# Autodesk Inventor assembly: WheelSuspension
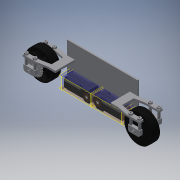
[picture p0: Inventor's stored thumbnail of the model, 180x180]
Saved by Autodesk Inventor 2017 (Build 210142000, 142)
## iProperties
Created: 2018-05-04
Part Number: WheelSuspension
Document SubType Name: Assembly
Designer: User
Author: User
## Documents named in this file (11)
- C:\Robotics\CAD\2018-19_CAD\Offseason\WheelSuspension.iam
- C:\Robotics\CAD\COTSParts\Fasteners\97345A207_316 STAINLESS STEEL SHOULDER SCREW.ipt
- C:\Robotics\CAD\COTSParts\Wheels\4in Wheel Intergreated Hub 8mm Rev2.ipt
- C:\Robotics\CAD\2016-17_CAD\Custom COTS\4inax.ipt
- C:\Robotics\CAD\2018-19_CAD\Offseason\WheelSuspensionHub.ipt
- C:\Robotics\CAD\COTSParts\Actobotics\535 parts\535198Bearing.25ID.5OD.ipt
- C:\Robotics\CAD\2018-19_CAD\Offseason\WheelandSprocketComboHub2.ipt
- C:\Robotics\CAD\COTSParts\Actobotics\615 parts\615106Sprocket.5inBore.25inPitch24Teeth.ipt
- C:\Robotics\CAD\2018-19_CAD\Offseason\WheelSuspensionFork.ipt
- C:\Robotics\CAD\2018-19_CAD\Offseason\SuspensionDrivePlate.ipt
- C:\Robotics\CAD\COTSParts\Rev\REV-41-1300HexMotor.ipt
## Components (30 placed, 10 different names)
1. 97345A207_316 STAINLESS STEEL SHOULDER SCREW:1 — Insert:3, Mate:3, Insert:11
2. 4in Wheel Intergreated Hub 8mm Rev2:1 — Insert:6
3. 4inax:1 — Insert:2
4. WheelSuspensionHub:1 — Insert:1, Insert:3, Mate:2, Insert:10
5. 535198Bearing.25ID.5OD:1 — Insert:1, Insert:2
6. WheelandSprocketComboHub2:1 — Insert:5, Insert:6, Insert:10
7. 615106Sprocket.5inBore.25inPitch24Teeth:1 — Insert:5
8. WheelSuspensionHub:2 — Insert:7, Insert:9
9. 97345A207_316 STAINLESS STEEL SHOULDER SCREW:2 — Insert:9, Mate:3, Insert:12
10. 535198Bearing.25ID.5OD:2 — Insert:7, Mate:2
11. WheelSuspensionFork:1 — Angle:1, Insert:11, Insert:12, Insert:13, Insert:14, Insert:27, Insert:28, Insert:31, Insert:34
12. 97345A207_316 STAINLESS STEEL SHOULDER SCREW:3 — Insert:13
13. 97345A207_316 STAINLESS STEEL SHOULDER SCREW:4 — Insert:14
14. 97345A207_316 STAINLESS STEEL SHOULDER SCREW:5
15. 4in Wheel Intergreated Hub 8mm Rev2:2
16. 4inax:2
17. WheelSuspensionHub:3
18. 535198Bearing.25ID.5OD:3
19. WheelandSprocketComboHub2:2
20. 615106Sprocket.5inBore.25inPitch24Teeth:2
21. WheelSuspensionHub:4
22. 97345A207_316 STAINLESS STEEL SHOULDER SCREW:6
23. 535198Bearing.25ID.5OD:4
24. WheelSuspensionFork:2 — Insert:29, Insert:30, Insert:32, Insert:33
25. 97345A207_316 STAINLESS STEEL SHOULDER SCREW:7
26. 97345A207_316 STAINLESS STEEL SHOULDER SCREW:8
27. SuspensionDrivePlate:1 — Insert:27, Insert:28, Insert:29, Insert:30
28. SuspensionDrivePlate:2 — Insert:31, Insert:32, Insert:33, Insert:34, Mate:6, Flush:1, Flush:2, Mate:7, Mate:8, Flush:3, Mate:10
29. REV-41-1300HexMotor:1 — Mate:8, Mate:9, Flush:3, Flush:4, Mate:10
30. REV-41-1300HexMotor:2 — Mate:7, Mate:9, Flush:4
## Relationships (46: Insert 32, Mate 9, Flush 4, Angle 1)
- Insert:1: WheelSuspensionHub:1 ↔ 535198Bearing.25ID.5OD:1
- Insert:2 (3.175 mm): 4inax:1 ↔ 535198Bearing.25ID.5OD:1
- Insert:3: 97345A207_316 STAINLESS STEEL SHOULDER SCREW:1 ↔ WheelSuspensionHub:1
- Insert:5: WheelandSprocketComboHub2:1 ↔ 615106Sprocket.5inBore.25inPitch24Teeth:1
- Insert:6: 4in Wheel Intergreated Hub 8mm Rev2:1 ↔ WheelandSprocketComboHub2:1
- Insert:7: WheelSuspensionHub:2 ↔ 535198Bearing.25ID.5OD:2
- Insert:9: WheelSuspensionHub:2 ↔ 97345A207_316 STAINLESS STEEL SHOULDER SCREW:2
- Mate:2: WheelSuspensionHub:1 ↔ 535198Bearing.25ID.5OD:2
- Mate:3 (63.5 mm): 97345A207_316 STAINLESS STEEL SHOULDER SCREW:1 ↔ 97345A207_316 STAINLESS STEEL SHOULDER SCREW:2
- Angle:1 (0 deg): WheelSuspensionFork:1
- Insert:10 (1.27 mm): WheelSuspensionHub:1 ↔ WheelandSprocketComboHub2:1
- Insert:11: 97345A207_316 STAINLESS STEEL SHOULDER SCREW:1 ↔ WheelSuspensionFork:1
- Insert:12: 97345A207_316 STAINLESS STEEL SHOULDER SCREW:2 ↔ WheelSuspensionFork:1
- Insert:13: WheelSuspensionFork:1 ↔ 97345A207_316 STAINLESS STEEL SHOULDER SCREW:3
- Insert:14: WheelSuspensionFork:1 ↔ 97345A207_316 STAINLESS STEEL SHOULDER SCREW:4
- [Insert]: WheelSuspensionHub:3 ↔ 535198Bearing.25ID.5OD:3
- [Insert] (3.175 mm): 4inax:2 ↔ 535198Bearing.25ID.5OD:3
- [Insert]: 97345A207_316 STAINLESS STEEL SHOULDER SCREW:5 ↔ WheelSuspensionHub:3
- [Insert]: WheelandSprocketComboHub2:2 ↔ 615106Sprocket.5inBore.25inPitch24Teeth:2
- [Insert]: 4in Wheel Intergreated Hub 8mm Rev2:2 ↔ WheelandSprocketComboHub2:2
- [Insert]: WheelSuspensionHub:4 ↔ 535198Bearing.25ID.5OD:4
- [Insert]: WheelSuspensionHub:4 ↔ 97345A207_316 STAINLESS STEEL SHOULDER SCREW:6
- [Mate]: WheelSuspensionHub:3 ↔ 535198Bearing.25ID.5OD:4
- [Mate] (63.5 mm): 97345A207_316 STAINLESS STEEL SHOULDER SCREW:5 ↔ 97345A207_316 STAINLESS STEEL SHOULDER SCREW:6
- [Insert] (1.27 mm): WheelSuspensionHub:3 ↔ WheelandSprocketComboHub2:2
- [Insert]: 97345A207_316 STAINLESS STEEL SHOULDER SCREW:5 ↔ WheelSuspensionFork:2
- [Insert]: 97345A207_316 STAINLESS STEEL SHOULDER SCREW:6 ↔ WheelSuspensionFork:2
- [Insert]: WheelSuspensionFork:2 ↔ 97345A207_316 STAINLESS STEEL SHOULDER SCREW:7
- [Insert]: WheelSuspensionFork:2 ↔ 97345A207_316 STAINLESS STEEL SHOULDER SCREW:8
- Insert:27: WheelSuspensionFork:1 ↔ SuspensionDrivePlate:1
- Insert:28: WheelSuspensionFork:1 ↔ SuspensionDrivePlate:1
- Insert:29: WheelSuspensionFork:2 ↔ SuspensionDrivePlate:1
- Insert:30: WheelSuspensionFork:2 ↔ SuspensionDrivePlate:1
- Insert:31: WheelSuspensionFork:1 ↔ SuspensionDrivePlate:2
- Insert:32: WheelSuspensionFork:2 ↔ SuspensionDrivePlate:2
- Insert:33: WheelSuspensionFork:2 ↔ SuspensionDrivePlate:2
- Insert:34: WheelSuspensionFork:1 ↔ SuspensionDrivePlate:2
- Mate:6: SuspensionDrivePlate:2
- Flush:1: SuspensionDrivePlate:2
- Flush:2: SuspensionDrivePlate:2
- Mate:7: SuspensionDrivePlate:2 ↔ REV-41-1300HexMotor:2
- Mate:8: SuspensionDrivePlate:2 ↔ REV-41-1300HexMotor:1
- Mate:9 (-3.175 mm): REV-41-1300HexMotor:1 ↔ REV-41-1300HexMotor:2
- Flush:3 (19.05 mm): SuspensionDrivePlate:2 ↔ REV-41-1300HexMotor:1
- Flush:4: REV-41-1300HexMotor:1 ↔ REV-41-1300HexMotor:2
- Mate:10: SuspensionDrivePlate:2 ↔ REV-41-1300HexMotor:1
## Named parameters: d22_d17 = 1.27 mm, d23_d18 = 0 mm, d24_d19 = 0 mm, d25_d20 = 0 mm, d26_d21 = 0 mm, d27_d0 = 0 mm, d28_d1 = 3.175 mm, d29_d2 = 0 mm, d30_d5 = 0 mm, d31_d6 = 0 mm, d32_d7 = 0 mm, d33_d9 = 0 mm, d34_d12 = 0 mm, d35_d14 = 63.5 mm
